# Autodesk Inventor assembly: Front_Panel_Base_Assembly
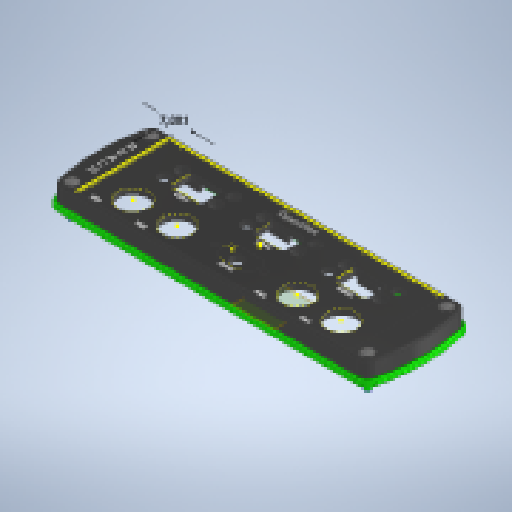
[picture p0: Inventor's stored thumbnail of the model, 512x512]
Saved by Autodesk Inventor 2024.2 (Build 282272000, 272)
## iProperties
Created: 2020-07-14
Part Number: Front_Panel_Base_Assembly
Document SubType Name: Assembly
Designer: CASE-SMALL2
Author: CASE-SMALL2
## Documents named in this file (8)
- C:\Users\lgnds\Documents\GitHub\REACH-Hardware\CAD\InventorProject\Front_Panel\Panel\Front_Panel_Base_Assembly.iam
- C:\Users\lgnds\Documents\GitHub\REACH-Hardware\CAD\InventorProject\Back_Panel\Panel\SHR Z KT30X10 WN 1452 OG_3DSYM.ipt
- C:\Users\lgnds\Documents\GitHub\REACH-Hardware\CAD\InventorProject\Back_Panel\Panel\1009410_3D.ipt
- C:\Users\lgnds\Documents\GitHub\REACH-Hardware\CAD\InventorProject\Front_Panel\Panel\1009799_3D_Front.ipt
- C:\Users\lgnds\Documents\GitHub\REACH-Hardware\CAD\InventorProject\Front_Panel\Panel\1009799_3D_Front_CAM_version.ipt
- C:\Users\lgnds\Documents\GitHub\REACH-Hardware\CAD\InventorProject\Front_Panel\Panel\1009799_3D_Front_WaveRunner.ipt
- C:\Users\lgnds\Documents\GitHub\REACH-Hardware\CAD\InventorProject\Back_Panel\Panel\DI 1600-6000.ipt
- C:\Users\lgnds\Documents\GitHub\REACH-Hardware\CAD\InventorProject\Front_Panel\Panel\1009799_3D_Front_10Gbit.ipt
## Components (13 placed, 7 different names)
1. 1009799_3D_Front:1 — Rigid:1, Rigid:2, Rigid:3, Rigid:4, Rigid:5, Rigid:6, Rigid:7, Rigid:8, Rigid:9, Rigid:11
2. 1009799_3D_Front_CAM_version:1 — Rigid:9
3. 1009799_3D_Front_WaveRunner:1
4. 1009799_3D_Front_10Gbit:1 — Rigid:11
5. DI 1600-6000:1
6. SHR Z KT30X10 WN 1452 OG_3DSYM:1 — Rigid:1
7. SHR Z KT30X10 WN 1452 OG_3DSYM:2 — Rigid:5
8. SHR Z KT30X10 WN 1452 OG_3DSYM:3 — Rigid:3
9. SHR Z KT30X10 WN 1452 OG_3DSYM:4 — Rigid:7
10. 1009410_3D:1 — Rigid:2
11. 1009410_3D:2 — Rigid:4
12. 1009410_3D:3 — Rigid:8
13. 1009410_3D:4 — Rigid:6
## Relationships (11: WeldJoint 11)
- Rigid:1 [WeldJoint]: 1009799_3D_Front:1 ↔ SHR Z KT30X10 WN 1452 OG_3DSYM:1
- Rigid:2 [WeldJoint]: 1009799_3D_Front:1 ↔ 1009410_3D:1
- Rigid:3 [WeldJoint]: 1009799_3D_Front:1 ↔ SHR Z KT30X10 WN 1452 OG_3DSYM:3
- Rigid:4 [WeldJoint]: 1009799_3D_Front:1 ↔ 1009410_3D:2
- Rigid:5 [WeldJoint]: 1009799_3D_Front:1 ↔ SHR Z KT30X10 WN 1452 OG_3DSYM:2
- Rigid:6 [WeldJoint]: 1009799_3D_Front:1 ↔ 1009410_3D:4
- Rigid:7 [WeldJoint]: 1009799_3D_Front:1 ↔ SHR Z KT30X10 WN 1452 OG_3DSYM:4
- Rigid:8 [WeldJoint]: 1009799_3D_Front:1 ↔ 1009410_3D:3
- Rigid:9 [WeldJoint]: 1009799_3D_Front:1 ↔ 1009799_3D_Front_CAM_version:1
- [WeldJoint]: 1009799_3D_Front_CAM_version:1 ↔ 1009799_3D_Front_WaveRunner:1
- Rigid:11 [WeldJoint]: 1009799_3D_Front:1 ↔ 1009799_3D_Front_10Gbit:1
